# Autodesk Inventor assembly: gate_valve_assembly
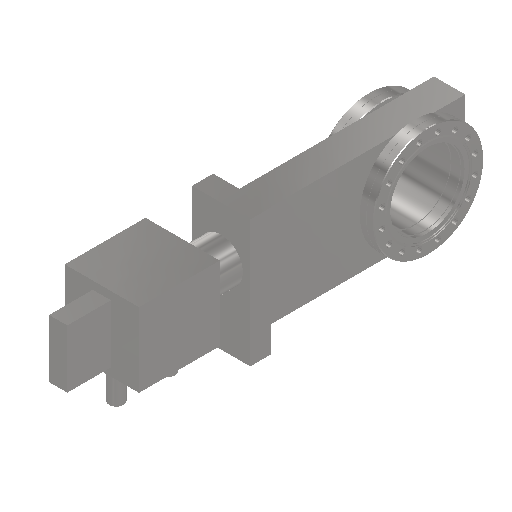
[picture p0: Inventor's stored thumbnail of the model, 512x512]
Saved by Autodesk Inventor 2026.2 (Build 302298000, 298)
## iProperties
Created: 2026-03-12
Part Number: gate_valve_assembly
Document SubType Name: Assembly
Designer: zetsu
Author: zetsu
## Documents named in this file (4)
- C:\Users\mzts1\OneDrive - Kyoto University\ドキュメント\蓮尾研究室\3D_CAD\parts\PHTI_1\parts\gate_valve\gate_valve_assembly.iam
- C:\Users\mzts1\OneDrive - Kyoto University\ドキュメント\蓮尾研究室\3D_CAD\parts\PHTI_1\parts\gate_valve\gate_valve.ipt
- C:\Users\mzts1\OneDrive - Kyoto University\ドキュメント\蓮尾研究室\3D_CAD\parts\PHTI_1\parts\gate_valve\UFC\UFC-152.ipt
- C:\Users\mzts1\OneDrive - Kyoto University\ドキュメント\蓮尾研究室\3D_CAD\parts\PHTI_1\parts\gate_valve\UFC.ipt
## Components (3 placed, 2 different names)
1. gate_valve:1 — メイト:1, メイト:2, メイト:3, メイト:4, 角度:1, 角度:2
2. UFC-152:1 — メイト:2, メイト:4, 角度:2
3. UFC-152:2 — メイト:1, メイト:3, 角度:1
## Relationships (6: Mate 4, Angle 2)
- メイト:1 [Mate]: gate_valve:1 ↔ UFC-152:2
- メイト:2 [Mate]: gate_valve:1 ↔ UFC-152:1
- メイト:3 [Mate]: gate_valve:1 ↔ UFC-152:2
- メイト:4 [Mate]: gate_valve:1 ↔ UFC-152:1
- 角度:1 [Angle] (0 deg): gate_valve:1 ↔ UFC-152:2
- 角度:2 [Angle] (0 deg): gate_valve:1 ↔ UFC-152:1
